# Autodesk Inventor assembly: Housing_Assembly
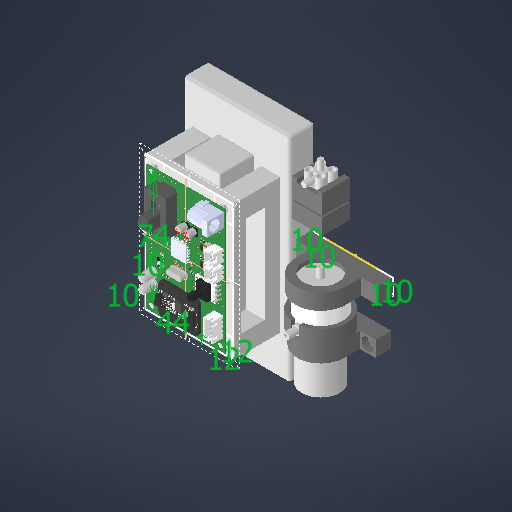
[picture p0: Inventor's stored thumbnail of the model, 512x512]
Saved by Autodesk Inventor 2026.2 (Build 302298000, 298)
## iProperties
Created: 2026-02-03
Part Number: Housing_Assembly
Document SubType Name: Assembly
Designer: vckot
Author: vckot
## iProperties of the stored document MemberDocs/x0iaocwioEc3obyvkEhahbepxYh
Created: 2026-02-03
Part Number: Housing_Assembly
Document SubType Name: Assembly
Designer: vckot
Author: vckot
## Documents named in this file (8)
- C:\Users\vckot\OneDrive\Documents\Vaibhav\capstone\CAD_files\Housing_Assembly.iam
- C:\Users\vckot\OneDrive\Documents\Vaibhav\capstone\CAD_files\PCB\TourniquetPCBV1_Updated\TourniquetPCBV1_Updated\TourniquetPCBV1_Updated.iam
- C:\Users\vckot\OneDrive\Documents\Vaibhav\capstone\CAD_files\Batteries\Battery_Small.ipt
- C:\Users\vckot\OneDrive\Documents\Vaibhav\capstone\CAD_files\PCB\PCB_Housing_01.ipt
- C:\Users\vckot\OneDrive\Documents\Vaibhav\capstone\CAD_files\Motor\Motor_Assembly.iam
- C:\Users\vckot\OneDrive\Documents\Vaibhav\capstone\CAD_files\Motor_Valve\Motor_Valve_Assembly.iam
- C:\Users\vckot\OneDrive\Documents\Vaibhav\capstone\CAD_files\Batteries\Battery_Large.ipt
- C:\Users\vckot\OneDrive\Documents\Vaibhav\capstone\CAD_files\PCB_Housing_02.ipt
## Components (7 placed, 7 different names)
1. TourniquetPCBV1_Updated:1 [sub-assembly] — Mate:1, Mate:2, Flush:1, Mate:3, Mate:4, Mate:6, Flush:6, Mate:8
2. Battery_Small:1 — Mate:1, Mate:2, Flush:1, Flush:2, Mate:5
3. PCB_Housing_01:1 — Mate:3, Mate:4, Flush:2, Flush:3
4. Motor_Assembly:1 [sub-assembly] — Flush:3, Mate:7
5. Motor_Valve_Assembly:1 [sub-assembly] — Mate:7
6. Battery_Large:1 — Mate:5, Mate:6, Flush:6, Flush:7
7. PCB_Housing_02:1 — Mate:8, Flush:7
## Relationships (13: Mate 8, Flush 5)
- Mate:1 (10 mm): TourniquetPCBV1_Updated:1 ↔ Battery_Small:1
- Mate:2: TourniquetPCBV1_Updated:1 ↔ Battery_Small:1
- Flush:1: TourniquetPCBV1_Updated:1 ↔ Battery_Small:1
- Mate:3: TourniquetPCBV1_Updated:1 ↔ PCB_Housing_01:1
- Mate:4: TourniquetPCBV1_Updated:1 ↔ PCB_Housing_01:1
- Flush:2: Battery_Small:1 ↔ PCB_Housing_01:1
- Flush:3: PCB_Housing_01:1 ↔ Motor_Assembly:1
- Mate:5: Battery_Small:1 ↔ Battery_Large:1
- Mate:6: TourniquetPCBV1_Updated:1 ↔ Battery_Large:1
- Flush:6: TourniquetPCBV1_Updated:1 ↔ Battery_Large:1
- Mate:7: Motor_Assembly:1 ↔ Motor_Valve_Assembly:1
- Mate:8 (20 mm): TourniquetPCBV1_Updated:1 ↔ PCB_Housing_02:1
- Flush:7 (-2 mm): Battery_Large:1 ↔ PCB_Housing_02:1
